# Autodesk Inventor assembly: lens-clamp-hsi
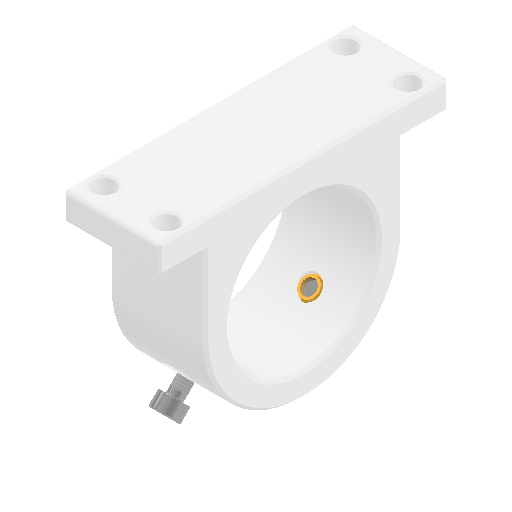
[picture p0: Inventor's stored thumbnail of the model, 512x512]
Saved by Autodesk Inventor 2026.2 (Build 302298000, 298)
## iProperties
Created: 2025-06-06
Part Number: lens-clamp-hsi
Document SubType Name: Assembly
Designer: kuzmin
Author: kuzmin
## Documents named in this file (4)
- D:\repos\PIHTI\LIBS\lens-clamp-hsi.iam
- D:\repos\PIHTI\LIBS\lens-clamp.ipt
- D:\repos\PIHTI\ContentCenter\Fastners\brass-insert-m3x5.ipt
- D:\repos\PIHTI\ContentCenter\Fastners\M3x8-SHCS.ipt
## Components (5 placed, 3 different names)
1. lens-clamp:1
2. brass-insert-m3x5:1 — メイト:1
3. brass-insert-m3x5:2 — メイト:2
4. SS ISO 4762 M3 x 8:1 — メイト:1
5. SS ISO 4762 M3 x 8:2 — メイト:2
## Relationships (4: WeldJoint 2, Mate 2)
- [WeldJoint]: lens-clamp:1 ↔ brass-insert-m3x5:1
- [WeldJoint]: lens-clamp:1 ↔ brass-insert-m3x5:2
- メイト:1 [Mate]: brass-insert-m3x5:1 ↔ SS ISO 4762 M3 x 8:1
- メイト:2 [Mate]: brass-insert-m3x5:2 ↔ SS ISO 4762 M3 x 8:2
